# Autodesk Inventor assembly: Assembly_USB_Lampassembly
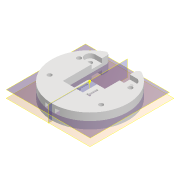
[picture p0: Inventor's stored thumbnail of the model, 180x180]
Saved by Autodesk Inventor 2022 (Build 260153000, 153)
## iProperties
Created: 2022-12-21
Part Number: Assembly_USB_Lampassembly
Document SubType Name: Assembly
Designer: diederichbenedict
Author: diederichbenedict
## Documents named in this file (3)
- C:\Users\diederichbenedict\Dropbox\Dokumente\Promotion\PROJECTS\Matchboxscope\INVENTOR\MATCHBOXSCOPE\Assembly_USB_Lampassembly.iam
- C:\Users\diederichbenedict\Dropbox\Dokumente\Promotion\PROJECTS\Matchboxscope\INVENTOR\MATCHBOXSCOPE\Matchboxscope_layer_ikealamp.ipt
- C:\Users\diederichbenedict\Dropbox\Dokumente\Promotion\PROJECTS\Matchboxscope\INVENTOR\Planktoscope_Mini\USB_dupont_Adapter.ipt
## Components (2 placed, 2 different names)
1. Matchboxscope_layer_ikealamp:1 — Passend:1
2. USB_dupont_Adapter:1 — Passend:1, Fluchtend:1
## Relationships (2: Mate 1, Flush 1)
- Passend:1 [Mate]: Matchboxscope_layer_ikealamp:1 ↔ USB_dupont_Adapter:1
- Fluchtend:1 [Flush] (-5 mm): USB_dupont_Adapter:1
